# Autodesk Inventor assembly: Assembly5
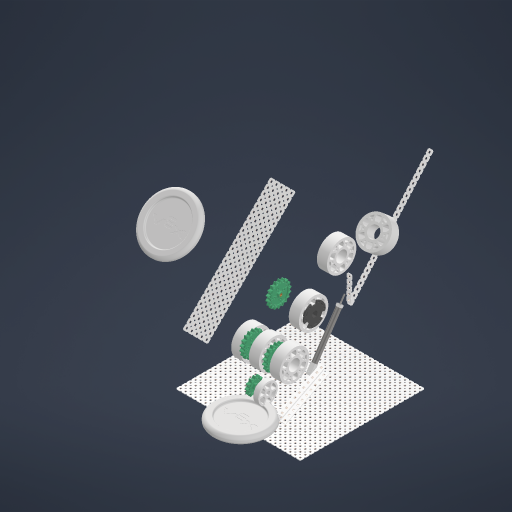
[picture p0: Inventor's stored thumbnail of the model, 512x512]
Saved by Autodesk Inventor 2023 (Build 270158000, 158)
## iProperties
Created: 2023-01-12
Part Number: Assembly5
Document SubType Name: Assembly
Designer: Windows Macbook
Author: Windows Macbook
## Documents named in this file (18)
- C:\Users\Windows Macbook\Desktop\Assembly5.iam
- C:\Users\Windows Macbook\Documents\Inventor\Content Center Files\VEX-CAD-Inventor-1.4.0\Structure\Plate\Aluminum\Alu Plate 25x25.iam
- C:\Users\Windows Macbook\Documents\Inventor\Content Center Files\VEX-CAD-Inventor-1.4.0\Motion\Wheels\Flex Wheels\2.000 Flex Wheel\2.000 30A .500.ipt
- C:\Users\Windows Macbook\Documents\Inventor\Content Center Files\VEX-CAD-Inventor-1.4.0\Motion\Wheels\Flex Wheels\2.000 Flex Wheel.ipt
- C:\Users\Windows Macbook\Documents\Inventor\Content Center Files\VEX-CAD-Inventor-1.4.0\Motion\Wheels\Flex Wheels\3.000 Flex Wheel\3.000 30A 1.000.ipt
- C:\Users\Windows Macbook\Documents\Inventor\Content Center Files\VEX-CAD-Inventor-1.4.0\Motion\Wheels\Flex Wheels\3.000 Flex Wheel.ipt
- C:\Users\Windows Macbook\Documents\Inventor\Content Center Files\276-7500-001 Web.ipt
- C:\Users\Windows Macbook\Documents\Inventor\Content Center Files\VEX-CAD-Inventor-1.4.0\Structure\Plate\Aluminum\Alu Plate 5x25.ipt
- C:\Users\Windows Macbook\Documents\Inventor\Content Center Files\VEX-CAD-Inventor-1.4.0\Structure\Plate\Aluminum\Alu Plate 1x5.ipt
- C:\Users\Windows Macbook\Documents\Inventor\Content Center Files\VEX-CAD-Inventor-1.4.0\Structure\Plate\Aluminum\Alu Plate 1x25.ipt
- C:\Users\Windows Macbook\Documents\Inventor\Content Center Files\VEX-CAD-Inventor-1.4.0\Motion\Pneumatics\Single Acting Piston.iam
- C:\Users\Windows Macbook\Documents\Inventor\Content Center Files\VEX-CAD-Inventor-1.4.0\Structure\C Channel\Aluminum 1x2x1\Alu C 1x2x1x10.ipt
- C:\Users\Windows Macbook\Documents\Inventor\Content Center Files\VEX-CAD-Inventor-1.4.0\Miscellaneous\Sizing Tool\VRC High School.ipt
- C:\Users\Windows Macbook\Documents\Inventor\Content Center Files\VEX-CAD-Inventor-1.4.0\Miscellaneous\Sizing Tool.ipt
- C:\Users\Windows Macbook\Documents\Inventor\Content Center Files\VEX-CAD-Inventor-1.4.0\Motion\Sprockets\9P Sprocket\9P 18T Sprocket, Circle.iam
- C:\Users\Windows Macbook\Documents\Inventor\Content Center Files\VEX-CAD-Inventor-1.4.0\Motion\Sprockets\9P Sprocket.iam
- C:\Users\Windows Macbook\Documents\Inventor\Content Center Files\VEX-CAD-Inventor-1.4.0\Motion\Sprockets\9P Sprocket\9P 12T Sprocket, Square.iam
- C:\Users\Windows Macbook\Documents\Inventor\Content Center Files\VEX-CAD-Inventor-1.4.0\Motion\Wheels\Flex Wheels\VersaHub.ipt
## Components (21 placed, 13 different names)
1. Alu Plate 25x25:1 [sub-assembly] — Flush:1, Angle:1, Mate:2
2. 2.000 30A .500:1
3. 276-7500-001 Web:1 — Mate:1
4. Alu Plate 5x25:1 — Mate:1, Angle:1, Mate:2
5. 3.000 30A 1.000:1
6. 3.000 30A 1.000:2 — Mate:3, Mate:4
7. Alu Plate 1x5:1
8. Alu Plate 1x25:1
9. Single Acting Piston:1 [sub-assembly]
10. 3.000 30A 1.000:3
11. 3.000 30A 1.000:4
12. 276-7500-001 Web:2
13. Alu C 1x2x1x10:1
14. VRC High School:1 — Flush:1
15. 3.000 30A 1.000:6
16. 3.000 30A 1.000:7
17. 9P 18T Sprocket, Circle:1 [sub-assembly]
18. 9P 12T Sprocket, Square:3 [sub-assembly]
19. 9P 18T Sprocket, Circle:4 [sub-assembly]
20. 9P 18T Sprocket, Circle:5 [sub-assembly]
21. VersaHub:1 — Mate:3, Mate:4
## Relationships (6: Mate 4, Flush 1, Angle 1)
- Mate:1: 276-7500-001 Web:1 ↔ Alu Plate 5x25:1
- Flush:1: Alu Plate 25x25:1 ↔ VRC High School:1
- Angle:1 (-45 deg): Alu Plate 25x25:1 ↔ Alu Plate 5x25:1
- Mate:2: Alu Plate 25x25:1 ↔ Alu Plate 5x25:1
- Mate:3: 3.000 30A 1.000:2 ↔ VersaHub:1
- Mate:4: 3.000 30A 1.000:2 ↔ VersaHub:1
